# Autodesk Inventor assembly: Slidey Mecanum L thing V2
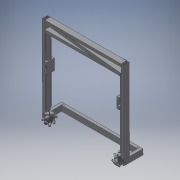
[picture p0: Inventor's stored thumbnail of the model, 180x180]
Saved by Autodesk Inventor 2018 (Build 220112000, 112)
## iProperties
Created: 2019-01-11
Part Number: Slidey Mecanum L thing V2
Document SubType Name: Assembly
Designer: s-2512711
Author: s-2512711
## Documents named in this file (9)
- \\studenthome\students\S-2512711\GitHub\2019CAD\Drivebase but Calvin is a mad man\Slidey Mecanum L thing V2.iam
- \\studenthome\students\S-2512711\GitHub\2019CAD\Drivebase but Calvin is a mad man\1X2 7in.ipt
- \\studenthome\students\S-2512711\GitHub\2019CAD\Drivebase but Calvin is a mad man\1x2 28in.ipt
- \\studenthome\students\S-2512711\GitHub\2019CAD\Drivebase but Calvin is a mad man\1x2 30in.ipt
- \\studenthome\students\S-2512711\GitHub\2019CAD\Drivebase but Calvin is a mad man\4_Mecanum_Wheel_Left_217-3644.iam
- \\studenthome\students\S-2512711\GitHub\2019CAD\Drivebase but Calvin is a mad man\4_Mecanum_Wheel_Right_217-3645.iam
- \\studenthome\students\S-2512711\GitHub\2019CAD\Drivebase but Calvin is a mad man\Strutural Integrity Bar.ipt
- \\studenthome\students\S-2512711\GitHub\2019CAD\Drivebase but Calvin is a mad man\Linear Guide Rail Temporary.ipt
- \\studenthome\students\S-2512711\GitHub\2019CAD\Drivebase but Calvin is a mad man\Temporary Guide.ipt
## Components (15 placed, 8 different names)
1. 1X2 7in:1 — Mate:4, Mate:5, Mate:6, Mate:7, Mate:8, Mate:9, Mate:22, Mate:23, Mate:24
2. 1X2 7in:2 — Mate:1, Mate:2, Mate:3, Mate:10, Mate:11, Mate:12, Mate:25, Mate:26, Mate:27
3. 1x2 28in:1 — Mate:7, Mate:8, Mate:9, Mate:10, Mate:11, Mate:12
4. 1x2 28in:2 — Mate:16, Mate:17, Flush:1, Mate:29, Mate:31
5. 1x2 28in:3 — Mate:13, Mate:14, Mate:15, Flush:1, Mate:18, Mate:19, Mate:20, Mate:21
6. 1x2 30in:1 — Mate:4, Mate:5, Mate:6, Mate:28, Flush:2
7. 1x2 30in:2 — Mate:1, Mate:2, Mate:3, Mate:13, Mate:14, Mate:15, Mate:16, Mate:17, Mate:30, Flush:3
8. 4_Mecanum_Wheel_Left_217-3644:1 [sub-assembly] — Mate:22, Mate:23, Mate:24
9. 4_Mecanum_Wheel_Right_217-3645:1 [sub-assembly] — Mate:25, Mate:26, Mate:27
10. Strutural Integrity Bar:1 — Mate:18, Mate:19
11. Strutural Integrity Bar:2 — Mate:20, Mate:21
12. Linear Guide Rail Temporary:1 — Mate:28, Mate:29, Flush:2, Mate:33, Flush:5
13. Linear Guide Rail Temporary:2 — Mate:30, Mate:31, Flush:3, Mate:32, Flush:4
14. Temporary Guide:1 — Mate:32, Flush:4
15. Temporary Guide:2 — Mate:33, Flush:5
## Relationships (38: Mate 33, Flush 5)
- Mate:1: 1X2 7in:2 ↔ 1x2 30in:2
- Mate:2: 1X2 7in:2 ↔ 1x2 30in:2
- Mate:3: 1X2 7in:2 ↔ 1x2 30in:2
- Mate:4: 1X2 7in:1 ↔ 1x2 30in:1
- Mate:5: 1X2 7in:1 ↔ 1x2 30in:1
- Mate:6: 1X2 7in:1 ↔ 1x2 30in:1
- Mate:7: 1X2 7in:1 ↔ 1x2 28in:1
- Mate:8: 1X2 7in:1 ↔ 1x2 28in:1
- Mate:9: 1X2 7in:1 ↔ 1x2 28in:1
- Mate:10: 1X2 7in:2 ↔ 1x2 28in:1
- Mate:11: 1X2 7in:2 ↔ 1x2 28in:1
- Mate:12: 1X2 7in:2 ↔ 1x2 28in:1
- Mate:13: 1x2 28in:3 ↔ 1x2 30in:2
- Mate:14: 1x2 28in:3 ↔ 1x2 30in:2
- Mate:15: 1x2 28in:3 ↔ 1x2 30in:2
- Mate:16: 1x2 28in:2 ↔ 1x2 30in:2
- Mate:17: 1x2 28in:2 ↔ 1x2 30in:2
- Flush:1 (76.2 mm): 1x2 28in:2 ↔ 1x2 28in:3
- Mate:18: 1x2 28in:3 ↔ Strutural Integrity Bar:1
- Mate:19: 1x2 28in:3 ↔ Strutural Integrity Bar:1
- Mate:20: 1x2 28in:3 ↔ Strutural Integrity Bar:2
- Mate:21: 1x2 28in:3 ↔ Strutural Integrity Bar:2
- Mate:22: 1X2 7in:1 ↔ 4_Mecanum_Wheel_Left_217-3644:1
- Mate:23: 1X2 7in:1 ↔ 4_Mecanum_Wheel_Left_217-3644:1
- Mate:24: 1X2 7in:1 ↔ 4_Mecanum_Wheel_Left_217-3644:1
- Mate:25: 1X2 7in:2 ↔ 4_Mecanum_Wheel_Right_217-3645:1
- Mate:26: 1X2 7in:2 ↔ 4_Mecanum_Wheel_Right_217-3645:1
- Mate:27: 1X2 7in:2 ↔ 4_Mecanum_Wheel_Right_217-3645:1
- Mate:28: 1x2 30in:1 ↔ Linear Guide Rail Temporary:1
- Mate:29: 1x2 28in:2 ↔ Linear Guide Rail Temporary:1
- Flush:2 (5.4864 mm): 1x2 30in:1 ↔ Linear Guide Rail Temporary:1
- Mate:30: 1x2 30in:2 ↔ Linear Guide Rail Temporary:2
- Mate:31: 1x2 28in:2 ↔ Linear Guide Rail Temporary:2
- Flush:3 (5.4864 mm): 1x2 30in:2 ↔ Linear Guide Rail Temporary:2
- Mate:32: Linear Guide Rail Temporary:2 ↔ Temporary Guide:1
- Flush:4 (-16.9164 mm): Linear Guide Rail Temporary:2 ↔ Temporary Guide:1
- Mate:33: Linear Guide Rail Temporary:1 ↔ Temporary Guide:2
- Flush:5 (-16.9164 mm): Linear Guide Rail Temporary:1 ↔ Temporary Guide:2
